# Autodesk Inventor assembly: ratchet
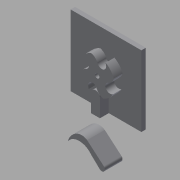
[picture p0: Inventor's stored thumbnail of the model, 180x180]
Saved by Autodesk Inventor 2013 (Build 170138000, 138)
## iProperties
Created: 2014-01-04
Part Number: ratchet
Document SubType Name: Assembly
Designer: kahohbein
Author: kahohbein
## Documents named in this file (5)
- C:\Users\kahohbein\Documents\GitHub\2013-2014_BlockParty\CAD\Lift\MK3\ratchet.iam
- C:\Users\kahohbein\Documents\GitHub\2013-2014_BlockParty\CAD\delete me\Part8.ipt
- C:\Users\kahohbein\Documents\GitHub\2013-2014_BlockParty\CAD\delete me\Part6.ipt
- C:\Users\kahohbein\Documents\GitHub\2013-2014_BlockParty\CAD\delete me\Part7.ipt
- C:\Users\kahohbein\Documents\GitHub\2013-2014_BlockParty\CAD\delete me\Part2.ipt
## Components (4 placed, 4 different names)
1. Part8:1 — Mate:1, Mate:2, Mate:3, Flush:1
2. Part6:1 — Mate:1, Mate:2
3. Part7:1 — Mate:3, Flush:1
4. Part2:1
## Relationships (4: Mate 3, Flush 1)
- Mate:1: Part8:1 ↔ Part6:1
- Mate:2: Part8:1 ↔ Part6:1
- Mate:3: Part8:1 ↔ Part7:1
- Flush:1: Part8:1 ↔ Part7:1
